# Autodesk Inventor assembly: Assy_fork_connection
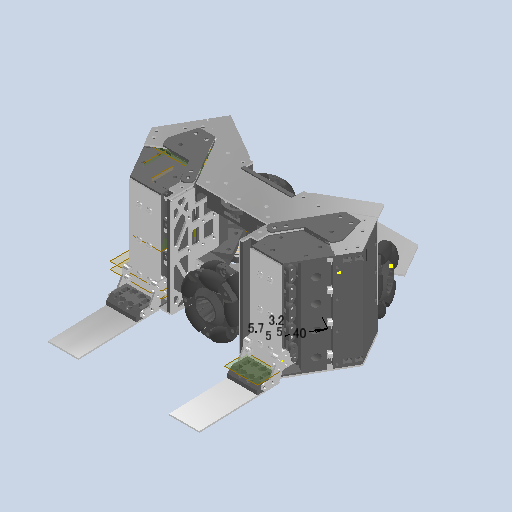
[picture p0: Inventor's stored thumbnail of the model, 512x512]
Saved by Autodesk Inventor 2024.1 (Build 281209000, 209)
## iProperties
Created: 2025-03-04
Part Number: Assy_fork_connection
Document SubType Name: Assembly
Designer: hibik
Author: hibik
## Documents named in this file (12)
- C:\Users\hibik\Documents\Robomech\RESCUE\ORCA\hard\Assy_fork_connection.iam
- C:\Users\hibik\Documents\Robomech\RESCUE\ORCA\hard\Assy_foot.iam
- C:\Users\hibik\Documents\Robomech\RESCUE\ORCA\hard\fork\right\Assy_fork_right.iam
- C:\Users\hibik\Documents\Robomech\RESCUE\ORCA\hard\flame_base\base2fork_connecter_front.ipt
- C:\Users\hibik\Documents\Robomech\RESCUE\ORCA\hard\flame_base\base2fork_connecter_back.ipt
- C:\Users\hibik\Documents\Robomech\RESCUE\ORCA\hard\fork\belt.ipt
- C:\Users\hibik\Documents\Robomech\RESCUE\ORCA\hard\fork\Assy_fork_left_test.iam
- C:\Users\hibik\Documents\Robomech\RESCUE\ORCA\hard\flame_base\upper_plate.ipt
- C:\Users\hibik\Documents\Robomech\RESCUE\ORCA\hard\fork\belt_geared_roller.ipt
- C:\Users\hibik\Documents\Robomech\RESCUE\ORCA\hard\fork\belt_roller_inside.ipt
- C:\Users\hibik\Documents\Robomech\RESCUE\ORCA\hard\fork\belt_roller_outside.ipt
- C:\Users\hibik\Documents\Robomech\RESCUE\ORCA\hard\fork\belt_cover_middle.ipt
## Components (16 placed, 11 different names)
1. Assy_foot:1 [sub-assembly] — 挿入:1, 挿入:2, 挿入:3, 挿入:4, 挿入:8, 挿入:9, 挿入:10, 挿入:11, 挿入:14, 角度:2
2. Assy_fork_right:1 [sub-assembly] — 挿入:5, 挿入:6, 挿入:7
3. base2fork_connecter_back:1 — 挿入:1, 挿入:2, 挿入:6
4. base2fork_connecter_front:1 — 挿入:3, 挿入:4, 挿入:5
5. belt:1 — 挿入:7, 角度:1
6. Assy_fork_left_test:1 [sub-assembly] — 挿入:12, 挿入:13
7. base2fork_connecter_front:2 — 挿入:10, 挿入:11, 挿入:12, 挿入:13
8. base2fork_connecter_back:2 — 挿入:8, 挿入:9
9. upper_plate:1 — 挿入:14, 角度:2, 挿入:18, 挿入:19, 挿入:20, メイト:1, メイト:2, フラッシュ:1
10. belt_geared_roller:1 — 挿入:17
11. belt_roller_inside:1 — 挿入:17, 挿入:20
12. belt_roller_inside:2 — 挿入:15, 挿入:18
13. belt_roller_inside:3 — 挿入:16, 挿入:19
14. belt_roller_outside:1 — 挿入:15
15. belt_roller_outside:2 — 挿入:16
16. belt_cover_middle:1 — メイト:1, メイト:2, フラッシュ:1
## Relationships (25: Insert 20, Angle 2, Mate 2, Flush 1)
- 挿入:1 [Insert]: Assy_foot:1 ↔ base2fork_connecter_back:1
- 挿入:2 [Insert]: Assy_foot:1 ↔ base2fork_connecter_back:1
- 挿入:3 [Insert]: Assy_foot:1 ↔ base2fork_connecter_front:1
- 挿入:4 [Insert]: Assy_foot:1 ↔ base2fork_connecter_front:1
- 挿入:5 [Insert]: Assy_fork_right:1 ↔ base2fork_connecter_front:1
- 挿入:6 [Insert]: Assy_fork_right:1 ↔ base2fork_connecter_back:1
- 挿入:7 [Insert]: Assy_fork_right:1 ↔ belt:1
- 角度:1 [Angle] (0 deg): belt:1
- 挿入:8 [Insert]: Assy_foot:1 ↔ base2fork_connecter_back:2
- 挿入:9 [Insert]: Assy_foot:1 ↔ base2fork_connecter_back:2
- 挿入:10 [Insert]: Assy_foot:1 ↔ base2fork_connecter_front:2
- 挿入:11 [Insert]: Assy_foot:1 ↔ base2fork_connecter_front:2
- 挿入:12 [Insert]: Assy_fork_left_test:1 ↔ base2fork_connecter_front:2
- 挿入:13 [Insert]: Assy_fork_left_test:1 ↔ base2fork_connecter_front:2
- 挿入:14 [Insert]: Assy_foot:1 ↔ upper_plate:1
- 角度:2 [Angle] (0 deg): Assy_foot:1 ↔ upper_plate:1
- 挿入:15 [Insert]: belt_roller_inside:2 ↔ belt_roller_outside:1
- 挿入:16 [Insert]: belt_roller_inside:3 ↔ belt_roller_outside:2
- 挿入:17 [Insert]: belt_geared_roller:1 ↔ belt_roller_inside:1
- 挿入:18 [Insert]: upper_plate:1 ↔ belt_roller_inside:2
- 挿入:19 [Insert]: upper_plate:1 ↔ belt_roller_inside:3
- 挿入:20 [Insert]: upper_plate:1 ↔ belt_roller_inside:1
- メイト:1 [Mate]: upper_plate:1 ↔ belt_cover_middle:1
- メイト:2 [Mate]: upper_plate:1 ↔ belt_cover_middle:1
- フラッシュ:1 [Flush]: upper_plate:1 ↔ belt_cover_middle:1
